# Autodesk Inventor assembly: xy-motion-assembly
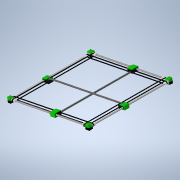
[picture p0: Inventor's stored thumbnail of the model, 180x180]
Saved by Autodesk Inventor 2020.4 (Build 244396000, 396)
## iProperties
Created: 2021-03-31
Part Number: xy-motion-assembly
Document SubType Name: Assembly
Designer: AOB
Mass: 1192.59 g
Surface Area: 2456.48 cm^2
Volume: 262.183 cm^3
Density: 4.5487 g/cm^3
Author: AOB
## Documents named in this file (11)
- C:\Users\marti\Documents\Inventor\ProjectBoron\Boron Ultima\xy-motion-assembly.iam
- C:\Users\marti\Documents\Inventor\ProjectBoron\Boron Ultima\xy-mount-assembly.iam
- C:\Users\marti\Documents\Inventor\ProjectBoron\Boron Ultima\8mm smooth rod.ipt
- C:\Users\marti\Documents\Inventor\ProjectBoron\Boron Ultima\xy-mount-assembly(right)1.iam
- C:\Users\marti\Documents\Inventor\ProjectBoron\Boron Ultima\double-head pulley.ipt
- C:\Users\marti\Documents\Inventor\ProjectBoron\Boron Ultima\xy-belt.ipt
- C:\Users\marti\Documents\Inventor\ProjectBoron\Boron Ultima\GT2 20T 6mm Powge-8mm bore.ipt
- C:\Users\marti\Documents\Inventor\ProjectBoron\Boron Ultima\f8-16 thrust bearing.ipt
- C:\Users\marti\Documents\Inventor\ProjectBoron\Boron Ultima\X-linear bearing shroud.iam
- C:\Users\marti\Documents\Inventor\ProjectBoron\Boron Ultima\Y-linear bearing shroud.iam
- C:\Users\marti\Documents\Inventor\ProjectBoron\Boron Ultima\8mm carbon fiber rod.ipt
## Components (34 placed, 10 different names)
1. 8mm smooth rod:1 — Rotational:1, Rotational:5, Mate:6, Angle:1, Mate:18, Cylindrical:2
2. 8mm smooth rod:2 — Rotational:4, Rotational:7, Mate:5, Mate:15, Angle:26, Cylindrical:1
3. 8mm smooth rod:3 — Rotational:2, Rotational:3, Mate:10, Mate:17, Cylindrical:4
4. 8mm smooth rod:4 — Mate:1, Mate:2, Mate:3, Mate:4, Mate:11, Angle:2, Mate:16, Cylindrical:3
5. xy-mount-assembly:1 [sub-assembly] — Rotational:1, Rotational:2, Mate:8, Mate:13, Rotational:14
6. xy-mount-assembly:2 [sub-assembly] — Rotational:7, Mate:2, Mate:3, Mate:21, Mate:23, Rotational:17, Rotational:18
7. xy-mount-assembly(mirror)1:1 [sub-assembly] — Rotational:3, Rotational:4, Mate:7, Mate:22, Rotational:15, Rotational:16
8. xy-mount-assembly(mirror)1:2 [sub-assembly] — Rotational:5, Mate:1, Mate:4, Mate:12, Mate:19, Mate:20, Rotational:11, Rotational:12
9. xy-belt:1 — Rotational:8, Mate:9
10. xy-belt:2 — Angle:1, Angle:2, Mate:25, Flush:1
11. xy-belt:3 — Rotational:10, Mate:24
12. xy-belt:4 — Rotational:9, Angle:26
13. double-head pulley:1 — Mate:5, Mate:7, Rotational:8
14. double-head pulley:2 — Mate:10, Mate:13, Mate:25, Flush:1
15. GT2 20T 6mm Powge-8mm bore:1 — Mate:6, Mate:8, Mate:9, Rotational:13
16. GT2 20T 6mm Powge-8mm bore:2 — Mate:11, Mate:12, Mate:20
17. GT2 20T 6mm Powge-8mm bore:3 — Mate:18, Mate:19, Mate:24
18. GT2 20T 6mm Powge-8mm bore:4 — Mate:16, Mate:23
19. GT2 20T 6mm Powge-8mm bore:5 — Mate:15, Mate:21, Rotational:10
20. GT2 20T 6mm Powge-8mm bore:6 — Mate:17, Mate:22, Rotational:9
21. f8-16 thrust bearing:1 — Rotational:18
22. f8-16 thrust bearing:2 — Rotational:15
23. f8-16 thrust bearing:3 — Rotational:16
24. f8-16 thrust bearing:4 — Rotational:17
25. f8-16 thrust bearing:5 — Rotational:14
26. f8-16 thrust bearing:6 — Rotational:13
27. f8-16 thrust bearing:7 — Rotational:12
28. f8-16 thrust bearing:8 — Rotational:11
29. X-linear bearing shroud:1 [sub-assembly] — Cylindrical:4, Mate:28
30. X-linear bearing shroud:2 [sub-assembly] — Cylindrical:3, Mate:27
31. Y-linear bearing shroud:1 [sub-assembly] — Cylindrical:1, Mate:26
32. Y-linear bearing shroud:2 [sub-assembly] — Cylindrical:2, Rigid:20
33. 8mm carbon fiber rod:1 — Rigid:20, Mate:26
34. 8mm carbon fiber rod:2 — Mate:27, Mate:28
## Relationships (53: Mate 27, RevoluteJoint 17, CylindricalJoint 4, Angle 3, Flush 1, WeldJoint 1)
- Rotational:1 [RevoluteJoint] (-5 mm): 8mm smooth rod:1 ↔ xy-mount-assembly:1
- Rotational:2 [RevoluteJoint] (5 mm): 8mm smooth rod:3 ↔ xy-mount-assembly:1
- Rotational:3 [RevoluteJoint] (5 mm): 8mm smooth rod:3 ↔ xy-mount-assembly(mirror)1:1
- Rotational:4 [RevoluteJoint] (5 mm): 8mm smooth rod:2 ↔ xy-mount-assembly(mirror)1:1
- Rotational:5 [RevoluteJoint] (5 mm): 8mm smooth rod:1 ↔ xy-mount-assembly(mirror)1:2
- Rotational:7 [RevoluteJoint] (-5 mm): 8mm smooth rod:2 ↔ xy-mount-assembly:2
- Mate:1: 8mm smooth rod:4 ↔ xy-mount-assembly(mirror)1:2
- Mate:2: 8mm smooth rod:4 ↔ xy-mount-assembly:2
- Mate:3 (-5 mm): 8mm smooth rod:4 ↔ xy-mount-assembly:2
- Mate:4 (-5 mm): 8mm smooth rod:4 ↔ xy-mount-assembly(mirror)1:2
- Mate:5: 8mm smooth rod:2 ↔ double-head pulley:1
- Mate:6: 8mm smooth rod:1 ↔ GT2 20T 6mm Powge-8mm bore:1
- Mate:7 (5 mm): xy-mount-assembly(mirror)1:1 ↔ double-head pulley:1
- Mate:8 (5 mm): xy-mount-assembly:1 ↔ GT2 20T 6mm Powge-8mm bore:1
- Rotational:8 [RevoluteJoint] (-0.5 mm): xy-belt:1 ↔ double-head pulley:1
- Mate:9: xy-belt:1 ↔ GT2 20T 6mm Powge-8mm bore:1
- Mate:10: 8mm smooth rod:3 ↔ double-head pulley:2
- Mate:11: 8mm smooth rod:4 ↔ GT2 20T 6mm Powge-8mm bore:2
- Mate:12 (5 mm): xy-mount-assembly(mirror)1:2 ↔ GT2 20T 6mm Powge-8mm bore:2
- Mate:13 (5 mm): xy-mount-assembly:1 ↔ double-head pulley:2
- Angle:1 (0 deg): 8mm smooth rod:1 ↔ xy-belt:2
- Angle:2 (0 deg): 8mm smooth rod:4 ↔ xy-belt:2
- Mate:15: 8mm smooth rod:2 ↔ GT2 20T 6mm Powge-8mm bore:5
- Mate:16: 8mm smooth rod:4 ↔ GT2 20T 6mm Powge-8mm bore:4
- Mate:17: 8mm smooth rod:3 ↔ GT2 20T 6mm Powge-8mm bore:6
- Mate:18: 8mm smooth rod:1 ↔ GT2 20T 6mm Powge-8mm bore:3
- Mate:19 (5 mm): xy-mount-assembly(mirror)1:2 ↔ GT2 20T 6mm Powge-8mm bore:3
- Mate:20 (5 mm): xy-mount-assembly(mirror)1:2 ↔ GT2 20T 6mm Powge-8mm bore:2
- Mate:21 (5 mm): xy-mount-assembly:2 ↔ GT2 20T 6mm Powge-8mm bore:5
- Mate:22 (5 mm): xy-mount-assembly(mirror)1:1 ↔ GT2 20T 6mm Powge-8mm bore:6
- Rotational:9 [RevoluteJoint] (-0.5 mm): xy-belt:4 ↔ GT2 20T 6mm Powge-8mm bore:6
- Mate:23 (5 mm): xy-mount-assembly:2 ↔ GT2 20T 6mm Powge-8mm bore:4
- Rotational:10 [RevoluteJoint] (-0.5 mm): xy-belt:3 ↔ GT2 20T 6mm Powge-8mm bore:5
- Mate:24: xy-belt:3 ↔ GT2 20T 6mm Powge-8mm bore:3
- Angle:26 (0 deg): 8mm smooth rod:2 ↔ xy-belt:4
- Mate:25: xy-belt:2 ↔ double-head pulley:2
- Flush:1 (6.5 mm): xy-belt:2 ↔ double-head pulley:2
- Rotational:11 [RevoluteJoint]: xy-mount-assembly(mirror)1:2 ↔ f8-16 thrust bearing:8
- Rotational:12 [RevoluteJoint]: xy-mount-assembly(mirror)1:2 ↔ f8-16 thrust bearing:7
- Rotational:13 [RevoluteJoint]: GT2 20T 6mm Powge-8mm bore:1 ↔ f8-16 thrust bearing:6
- Rotational:14 [RevoluteJoint]: xy-mount-assembly:1 ↔ f8-16 thrust bearing:5
- Rotational:15 [RevoluteJoint]: xy-mount-assembly(mirror)1:1 ↔ f8-16 thrust bearing:2
- Rotational:16 [RevoluteJoint]: xy-mount-assembly(mirror)1:1 ↔ f8-16 thrust bearing:3
- Rotational:17 [RevoluteJoint]: xy-mount-assembly:2 ↔ f8-16 thrust bearing:4
- Rotational:18 [RevoluteJoint]: xy-mount-assembly:2 ↔ f8-16 thrust bearing:1
- Cylindrical:1: 8mm smooth rod:2 ↔ Y-linear bearing shroud:1
- Cylindrical:2: 8mm smooth rod:1 ↔ Y-linear bearing shroud:2
- Cylindrical:3: 8mm smooth rod:4 ↔ X-linear bearing shroud:2
- Cylindrical:4: 8mm smooth rod:3 ↔ X-linear bearing shroud:1
- Rigid:20 [WeldJoint] (-13.4 mm): Y-linear bearing shroud:2 ↔ 8mm carbon fiber rod:1
- Mate:26: Y-linear bearing shroud:1 ↔ 8mm carbon fiber rod:1
- Mate:27: X-linear bearing shroud:2 ↔ 8mm carbon fiber rod:2
- Mate:28: X-linear bearing shroud:1 ↔ 8mm carbon fiber rod:2
